# Autodesk Inventor assembly: Mind
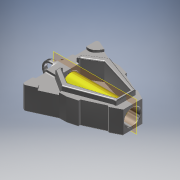
[picture p0: Inventor's stored thumbnail of the model, 180x180]
Saved by Autodesk Inventor 2019 (Build 230136000, 136)
## iProperties
Created: 2019-05-15
Part Number: Mind
Document SubType Name: Assembly
Designer: Jorian Brusind
Author: Jorian Brusind
## Documents named in this file (3)
- C:\Users\Jorian Brusind\Documents\GitHub\PersonalProjects\Inventor Projects\Infinity\Mind.iam
- C:\Users\Jorian Brusind\Documents\GitHub\PersonalProjects\Inventor Projects\Infinity\Yellow.ipt
- C:\Users\Jorian Brusind\Documents\GitHub\PersonalProjects\Inventor Projects\Infinity\Holder.ipt
## Components (2 placed, 2 different names)
1. Yellow:1 — Mate:1, Mate:2
2. Holder:1 — Mate:1, Mate:2
## Relationships (2: Mate 2)
- Mate:1: Yellow:1 ↔ Holder:1
- Mate:2: Yellow:1 ↔ Holder:1
